# Autodesk Inventor assembly: Baugruppe1
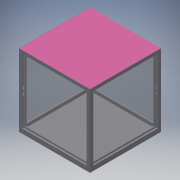
[picture p0: Inventor's stored thumbnail of the model, 180x180]
Saved by Autodesk Inventor 2018.3 (Build 223284000, 284)
## iProperties
Created: 2019-09-20
Part Number: Baugruppe1
Material: Generisch
Document SubType Name: Assembly
Designer: Lolob
Author: Lolob
## Documents named in this file (11)
- D:\Dokumente\S ch u l e\Dipl\Smartcube_Construction\Version_3\Baugruppe1.iam
- D:\Dokumente\S ch u l e\Dipl\Smartcube_Construction\Version_2\PV_Ramen_CPY_3.ipt
- D:\Dokumente\S ch u l e\Dipl\Smartcube_Construction\Version_2\PV_Modul_CPY_3.ipt
- D:\Dokumente\S ch u l e\Dipl\Smartcube_Construction\Version_3\Boden.ipt
- D:\Dokumente\S ch u l e\Dipl\Smartcube_Construction\Version_2\PV_Ramen_CPY_3_CPY.ipt
- D:\Dokumente\S ch u l e\Dipl\Smartcube_Construction\Version_2\PV_Modul_CPY_3_CPY.ipt
- D:\Dokumente\S ch u l e\Dipl\Smartcube_Construction\Version_2\PV_Ramen_CPY_3_CPY1.ipt
- D:\Dokumente\S ch u l e\Dipl\Smartcube_Construction\Version_2\PV_Modul_CPY_3_CPY1.ipt
- D:\Dokumente\S ch u l e\Dipl\Smartcube_Construction\Version_2\PV_Ramen_CPY_3_CPY2.ipt
- D:\Dokumente\S ch u l e\Dipl\Smartcube_Construction\Version_2\PV_Modul_CPY_3_CPY2.ipt
- D:\Dokumente\Inventor\Projektname\Boden_2.ipt
## Components (10 placed, 10 different names)
1. Boden:1 — Starr:5, Starr:9, Starr:10, Starr:11
2. PV_Ramen_CPY_3:1 — Starr:4, Drehbar:1, Starr:5
3. PV_Modul_CPY_3:1 — Starr:4, Drehbar:1
4. PV_Ramen_CPY_3_CPY:1 — Drehbar:2, Starr:6, Starr:10, Starr:12
5. PV_Modul_CPY_3_CPY:1 — Drehbar:2, Starr:6
6. PV_Ramen_CPY_3_CPY1:1 — Drehbar:3, Starr:7, Starr:9
7. PV_Modul_CPY_3_CPY1:1 — Drehbar:3, Starr:7
8. PV_Ramen_CPY_3_CPY2:1 — Drehbar:4, Starr:8, Starr:11
9. PV_Modul_CPY_3_CPY2:1 — Drehbar:4, Starr:8
10. Boden_2:1 — Fluchtend:1, Starr:12
## Relationships (14: WeldJoint 9, RevoluteJoint 4, Flush 1)
- Starr:4 [WeldJoint]: PV_Ramen_CPY_3:1 ↔ PV_Modul_CPY_3:1
- Drehbar:1 [RevoluteJoint]: PV_Ramen_CPY_3:1 ↔ PV_Modul_CPY_3:1
- Starr:5 [WeldJoint]: Boden:1 ↔ PV_Ramen_CPY_3:1
- Drehbar:2 [RevoluteJoint]: PV_Ramen_CPY_3_CPY:1 ↔ PV_Modul_CPY_3_CPY:1
- Starr:6 [WeldJoint]: PV_Ramen_CPY_3_CPY:1 ↔ PV_Modul_CPY_3_CPY:1
- Drehbar:3 [RevoluteJoint]: PV_Ramen_CPY_3_CPY1:1 ↔ PV_Modul_CPY_3_CPY1:1
- Starr:7 [WeldJoint]: PV_Ramen_CPY_3_CPY1:1 ↔ PV_Modul_CPY_3_CPY1:1
- Drehbar:4 [RevoluteJoint]: PV_Ramen_CPY_3_CPY2:1 ↔ PV_Modul_CPY_3_CPY2:1
- Starr:8 [WeldJoint]: PV_Ramen_CPY_3_CPY2:1 ↔ PV_Modul_CPY_3_CPY2:1
- Starr:9 [WeldJoint]: Boden:1 ↔ PV_Ramen_CPY_3_CPY1:1
- Starr:10 [WeldJoint]: Boden:1 ↔ PV_Ramen_CPY_3_CPY:1
- Starr:11 [WeldJoint]: Boden:1 ↔ PV_Ramen_CPY_3_CPY2:1
- Fluchtend:1 [Flush]: Boden_2:1
- Starr:12 [WeldJoint]: PV_Ramen_CPY_3_CPY:1 ↔ Boden_2:1
